# Autodesk Inventor assembly: Assembly1
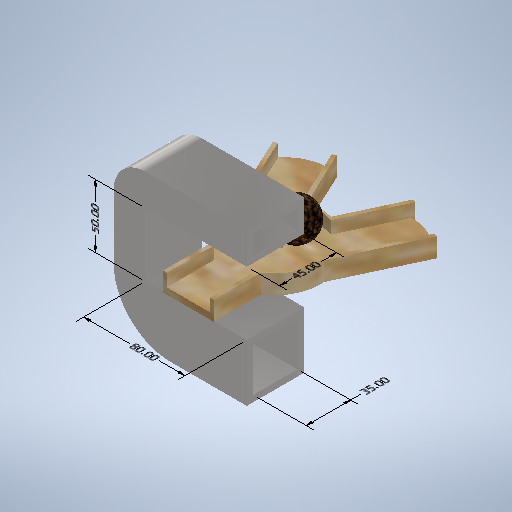
[picture p0: Inventor's stored thumbnail of the model, 512x512]
Saved by Autodesk Inventor 2025.4 (Build 294407000, 407)
## iProperties
Created: 2026-03-03
Part Number: Assembly1
Document SubType Name: Assembly
Designer: Amir
Author: Amir
## Documents named in this file (5)
- E:\omar\spring 26\Basics of Mechatronics\Assembly1.iam
- E:\omar\spring 26\Basics of Mechatronics\Part2.ipt
- E:\omar\spring 26\Basics of Mechatronics\Part1.ipt
- E:\omar\spring 26\Basics of Mechatronics\Part4.ipt
- E:\omar\spring 26\Basics of Mechatronics\pin 2.ipt
## Components (4 placed, 4 different names)
1. Part1:1
2. Part2:2 — Mate:1
3. Part4:1 — Mate:1, Mate:2, Mate:3
4. pin 2:1 — Mate:2, Mate:3
## Relationships (3: Mate 3)
- Mate:1: Part2:2 ↔ Part4:1
- Mate:2: Part4:1 ↔ pin 2:1
- Mate:3: Part4:1 ↔ pin 2:1
